# Autodesk Inventor assembly: groundStation-assy
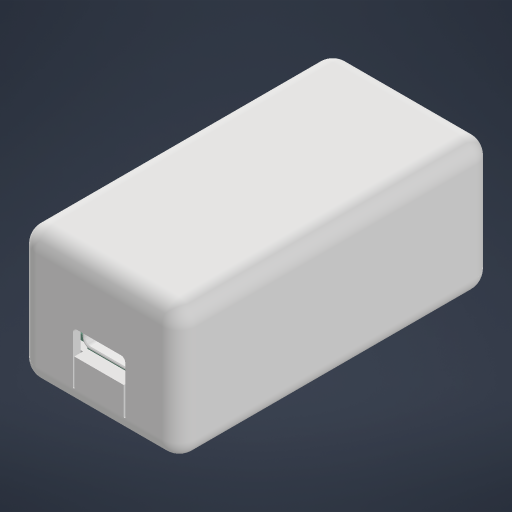
[picture p0: Inventor's stored thumbnail of the model, 512x512]
Saved by Autodesk Inventor 2024 (Build 280153000, 153)
## iProperties
Created: 2024-02-06
Part Number: groundStation-assy
Document SubType Name: Assembly
Designer: madis
Author: madis
## Documents named in this file (4)
- D:\Destination-SPACE-Files\development\hardware\groundStation\groundStation-assy.iam
- D:\Destination-SPACE-Files\development\hardware\groundStation\groundStation-Bottom.ipt
- D:\Destination-SPACE-Files\development\hardware\groundStation\groundStation-top.ipt
- D:\Destination-SPACE-Files\development\hardware\groundStation\esp32s3-main\esp32s3-main\3d models\FeatherS3\FeatherS3_uFL\FeatherS3_uFL.iam
## Components (3 placed, 3 different names)
1. groundStation-Bottom:1 — Mate:1, Mate:2, Mate:3, Mate:4, Mate:5, Mate:6, Mate:7
2. groundStation-top:1 — Mate:5, Mate:6, Mate:7
3. FeatherS3_uFL:1 [sub-assembly] — Mate:1, Mate:2, Mate:3, Mate:4
## Relationships (7: Mate 7)
- Mate:1: groundStation-Bottom:1 ↔ FeatherS3_uFL:1
- Mate:2: groundStation-Bottom:1 ↔ FeatherS3_uFL:1
- Mate:3: groundStation-Bottom:1 ↔ FeatherS3_uFL:1
- Mate:4: groundStation-Bottom:1 ↔ FeatherS3_uFL:1
- Mate:5: groundStation-Bottom:1 ↔ groundStation-top:1
- Mate:6: groundStation-Bottom:1 ↔ groundStation-top:1
- Mate:7: groundStation-Bottom:1 ↔ groundStation-top:1
